# Autodesk Inventor assembly: Expansor
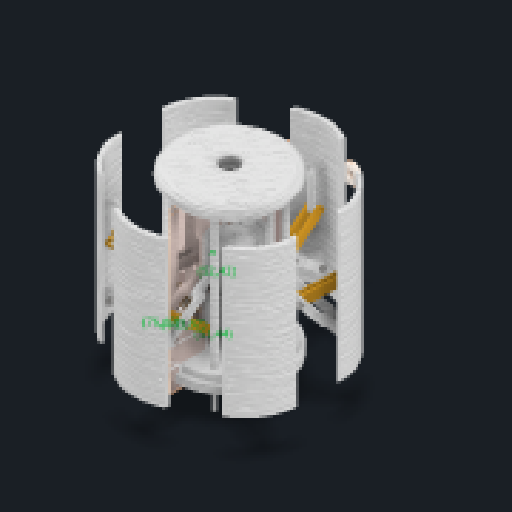
[picture p0: Inventor's stored thumbnail of the model, 512x512]
Saved by Autodesk Inventor 2025.3 (Build 293356030, 356C)
## iProperties
Created: 2024-12-25
Part Number: Expansor
Document SubType Name: Assembly
Designer: Usuario
Mass: 1399.4 g
Surface Area: 2444.05 cm^2
Volume: 493.018 cm^3
Density: 2.83844 g/cm^3
Author: Usuario
## Documents named in this file (19)
- C:\Users\santa\OneDrive - Universidad de los Andes\Robocol\Flotador\V3\Expansor.iam
- C:\Users\santa\OneDrive - Universidad de los Andes\Robocol\Flotador\V3\Expansor\Clavija.ipt
- C:\Users\santa\OneDrive - Universidad de los Andes\Robocol\Flotador\V3\Expansor\Columnas.ipt
- C:\Users\santa\OneDrive - Universidad de los Andes\Robocol\Flotador\V3\Expansor\Corredera I.ipt
- C:\Users\santa\OneDrive - Universidad de los Andes\Robocol\Flotador\V3\Expansor\Corredera II.ipt
- C:\Users\santa\OneDrive - Universidad de los Andes\Robocol\Flotador\V3\Expansor\Corredor.ipt
- C:\Users\santa\OneDrive - Universidad de los Andes\Robocol\Flotador\V3\Expansor\Paletas.ipt
- C:\Users\santa\OneDrive - Universidad de los Andes\Robocol\Flotador\V3\Expansor\Soporte.ipt
- C:\Users\santa\OneDrive - Universidad de los Andes\Robocol\Flotador\V3\Expansor\Tapa.ipt
- C:\Users\santa\OneDrive - Universidad de los Andes\Robocol\Flotador\Downloads\screw nut 8mm\screw nut 8mm.ipt
- C:\Users\santa\OneDrive\Documents\Inventor\Content Center Files\R2025\es-ES\ANSI B18.16.3M(2)\ANSI B18.16.3M - Property Class 5 and 10 - Metric M3 x 0.5 Tipo de metal.ipt
- C:\Users\santa\OneDrive\Documents\Inventor\Content Center Files\R2025\es-ES\AS 1420\AS 1420 - 1973 - M3 x 16.ipt
- C:\Users\santa\OneDrive - Universidad de los Andes\Robocol\Flotador\Downloads\688zz-bearing-2.snapshot.2\688ZZ Bearing\688ZZ Bearing Assembly\688ZZ Bearing Assembly\688ZZ Bearing Assembly.iam
- C:\Users\santa\OneDrive - Universidad de los Andes\Robocol\Flotador\V3\Expansor\AIP\FEA\exazi096o.fins
- C:\Users\santa\OneDrive - Universidad de los Andes\Robocol\Flotador\V3\Expansor\AIP\FEA\exazi096o.fsat
- C:\Users\santa\OneDrive - Universidad de los Andes\Robocol\Flotador\V3\Expansor\AIP\FEA\exazi096o.ftes
- C:\Users\santa\OneDrive - Universidad de los Andes\Robocol\Flotador\V3\Expansor\AIP\FEA\exazi096o.fwiz
- C:\Users\santa\OneDrive - Universidad de los Andes\Robocol\Flotador\V3\Expansor\AIP\FEA\exazi09pc.fmsh
- C:\Users\santa\OneDrive - Universidad de los Andes\Robocol\Flotador\V3\Expansor\AIP\FEA\exazi09pd.fres
## Components (83 placed, 12 different names)
1. Corredor:1 — ANIMAR, De rotación:5, Rígido:3, Simetría:1, Coincidencia:5, Simetría:2
2. Soporte:1 — Nivelación:1, Coincidencia:1, Nivelación:2, Rígido:1, ANIMAR, De rotación:3, Simetría:1, Simetría:2
3. Tapa:1 — Coincidencia:34, De rotación:6, Coincidencia:35
4. screw nut 8mm:1 — Rígido:3
5. 688ZZ Bearing Assembly:1 [sub-assembly] — De rotación:6
6. Tuerca hexagonal autofrenada - Acero Métrico Property Class 5 and 10 - Metric M3 x 0.5 Tipo de metal:2 — Coincidencia:10, Coincidencia:11
7. Tuerca hexagonal autofrenada - Acero Métrico Property Class 5 and 10 - Metric M3 x 0.5 Tipo de metal:4 — Coincidencia:28, Coincidencia:29
8. Tuerca hexagonal autofrenada - Acero Métrico Property Class 5 and 10 - Metric M3 x 0.5 Tipo de metal:3 — Coincidencia:14, Coincidencia:15
9. AS 1420 - Métrico M3 x 16:3 — Coincidencia:12, Coincidencia:13
10. AS 1420 - Métrico M3 x 16:4 — Coincidencia:26, Coincidencia:27
11. Tuerca hexagonal autofrenada - Acero Métrico Property Class 5 and 10 - Metric M3 x 0.5 Tipo de metal:5 — Coincidencia:32, Coincidencia:33
12. AS 1420 - Métrico M3 x 16:2 — Coincidencia:30, Coincidencia:31
13. Tuerca hexagonal autofrenada - Acero Métrico Property Class 5 and 10 - Metric M3 x 0.5 Tipo de metal:1 — Insertar:1
14. Columnas:1 — Rígido:1, Coincidencia:35
15. Corredera II:1 — De rotación:3, Coincidencia:3, Tangente:1, Coincidencia:7, Coincidencia:8, Coincidencia:9, Coincidencia:26, Coincidencia:27, Coincidencia:28, Coincidencia:29
16. Corredera I:1 — De rotación:5, Coincidencia:3, Coincidencia:6, Insertar:1, Coincidencia:11, Coincidencia:12, Coincidencia:13, Coincidencia:14, Coincidencia:15, Coincidencia:30, Coincidencia:31, Coincidencia:32, Coincidencia:33
17. Paletas:1 — Coincidencia:6, Tangente:1, Coincidencia:7
18. Clavija:1 — Coincidencia:8, Coincidencia:9, Coincidencia:10
19. Tuerca hexagonal autofrenada - Acero Métrico Property Class 5 and 10 - Metric M3 x 0.5 Tipo de metal:6
20. Tuerca hexagonal autofrenada - Acero Métrico Property Class 5 and 10 - Metric M3 x 0.5 Tipo de metal:7
21. Tuerca hexagonal autofrenada - Acero Métrico Property Class 5 and 10 - Metric M3 x 0.5 Tipo de metal:8
22. AS 1420 - Métrico M3 x 16:5
23. AS 1420 - Métrico M3 x 16:6
24. Tuerca hexagonal autofrenada - Acero Métrico Property Class 5 and 10 - Metric M3 x 0.5 Tipo de metal:9
25. AS 1420 - Métrico M3 x 16:7
26. Tuerca hexagonal autofrenada - Acero Métrico Property Class 5 and 10 - Metric M3 x 0.5 Tipo de metal:10
27. Columnas:2
28. Corredera II:2
29. Corredera I:2
30. Paletas:2
31. Clavija:2
32. Tuerca hexagonal autofrenada - Acero Métrico Property Class 5 and 10 - Metric M3 x 0.5 Tipo de metal:11
33. Tuerca hexagonal autofrenada - Acero Métrico Property Class 5 and 10 - Metric M3 x 0.5 Tipo de metal:12
34. Tuerca hexagonal autofrenada - Acero Métrico Property Class 5 and 10 - Metric M3 x 0.5 Tipo de metal:13
35. AS 1420 - Métrico M3 x 16:8
36. AS 1420 - Métrico M3 x 16:9
37. Tuerca hexagonal autofrenada - Acero Métrico Property Class 5 and 10 - Metric M3 x 0.5 Tipo de metal:14
38. AS 1420 - Métrico M3 x 16:10
39. Tuerca hexagonal autofrenada - Acero Métrico Property Class 5 and 10 - Metric M3 x 0.5 Tipo de metal:15
40. Columnas:3
41. Corredera II:3
42. Corredera I:3
43. Paletas:3
44. Clavija:3
45. Tuerca hexagonal autofrenada - Acero Métrico Property Class 5 and 10 - Metric M3 x 0.5 Tipo de metal:16
46. Tuerca hexagonal autofrenada - Acero Métrico Property Class 5 and 10 - Metric M3 x 0.5 Tipo de metal:17
47. Tuerca hexagonal autofrenada - Acero Métrico Property Class 5 and 10 - Metric M3 x 0.5 Tipo de metal:18
48. AS 1420 - Métrico M3 x 16:11
49. AS 1420 - Métrico M3 x 16:12
50. Tuerca hexagonal autofrenada - Acero Métrico Property Class 5 and 10 - Metric M3 x 0.5 Tipo de metal:19
51. AS 1420 - Métrico M3 x 16:13
52. Tuerca hexagonal autofrenada - Acero Métrico Property Class 5 and 10 - Metric M3 x 0.5 Tipo de metal:20
53. Columnas:4
54. Corredera II:4
55. Corredera I:4
56. Paletas:4
57. Clavija:4
58. Tuerca hexagonal autofrenada - Acero Métrico Property Class 5 and 10 - Metric M3 x 0.5 Tipo de metal:21
59. Tuerca hexagonal autofrenada - Acero Métrico Property Class 5 and 10 - Metric M3 x 0.5 Tipo de metal:22
60. Tuerca hexagonal autofrenada - Acero Métrico Property Class 5 and 10 - Metric M3 x 0.5 Tipo de metal:23
61. AS 1420 - Métrico M3 x 16:14
62. AS 1420 - Métrico M3 x 16:15
63. Tuerca hexagonal autofrenada - Acero Métrico Property Class 5 and 10 - Metric M3 x 0.5 Tipo de metal:24
64. AS 1420 - Métrico M3 x 16:16
65. Tuerca hexagonal autofrenada - Acero Métrico Property Class 5 and 10 - Metric M3 x 0.5 Tipo de metal:25
66. Columnas:5
67. Corredera II:5
68. Corredera I:5
69. Paletas:5
70. Clavija:5
71. Tuerca hexagonal autofrenada - Acero Métrico Property Class 5 and 10 - Metric M3 x 0.5 Tipo de metal:26
72. Tuerca hexagonal autofrenada - Acero Métrico Property Class 5 and 10 - Metric M3 x 0.5 Tipo de metal:27
73. Tuerca hexagonal autofrenada - Acero Métrico Property Class 5 and 10 - Metric M3 x 0.5 Tipo de metal:28
74. AS 1420 - Métrico M3 x 16:17
75. AS 1420 - Métrico M3 x 16:18
76. Tuerca hexagonal autofrenada - Acero Métrico Property Class 5 and 10 - Metric M3 x 0.5 Tipo de metal:29
77. AS 1420 - Métrico M3 x 16:19
78. Tuerca hexagonal autofrenada - Acero Métrico Property Class 5 and 10 - Metric M3 x 0.5 Tipo de metal:30
79. Columnas:6
80. Corredera II:6
81. Corredera I:6
82. Paletas:6
83. Clavija:6
## Component patterns: (6 elements, first: Tuerca hexagonal autofrenada - Acero Métrico Property Class 5 and 10 - Metric M3 x 0.5 Tipo de metal:2 + Tuerca hexagonal autofrenada - Acero Métrico Property Class 5 and 10 - Metric M3 x 0.5 Tipo de metal:4 + Tuerca hexagonal autofrenada - Acero Métrico Property Class 5 and 10 - Metric M3 x 0.5 Tipo de metal:3 + AS 1420 - Métrico M3 x 16:3 + AS 1420 - Métrico M3 x 16:4 + Tuerca hexagonal autofrenada - Acero Métrico Property Class 5 and 10 - Metric M3 x 0.5 Tipo de metal:5 + AS 1420 - Métrico M3 x 16:2 + Tuerca hexagonal autofrenada - Acero Métrico Property Class 5 and 10 - Metric M3 x 0.5 Tipo de metal:1 + Columnas:1 + Corredera II:1 + Corredera I:1 + Paletas:1 + Clavija:1)
## Relationships (35: Mate 23, RevoluteJoint 3, Flush 2, WeldJoint 2, Symmetry 2, CylindricalJoint 1, Tangent 1, Insert 1)
- Nivelación:1 [Flush]: Soporte:1
- Coincidencia:1 [Mate]: Soporte:1
- Nivelación:2 [Flush]: Soporte:1
- Rígido:1 [WeldJoint]: Soporte:1 ↔ Columnas:1
- ANIMAR [CylindricalJoint]: Corredor:1 ↔ Soporte:1
- De rotación:3 [RevoluteJoint]: Soporte:1 ↔ Corredera II:1
- De rotación:5 [RevoluteJoint]: Corredor:1 ↔ Corredera I:1
- Rígido:3 [WeldJoint]: Corredor:1 ↔ screw nut 8mm:1
- Simetría:1 [Symmetry]: Corredor:1 ↔ Soporte:1
- Coincidencia:3 [Mate]: Corredera II:1 ↔ Corredera I:1
- Coincidencia:5 [Mate]: Corredor:1
- Simetría:2 [Symmetry]: Corredor:1 ↔ Soporte:1
- Coincidencia:6 [Mate]: Corredera I:1 ↔ Paletas:1
- Tangente:1: Corredera II:1 ↔ Paletas:1
- Coincidencia:7 [Mate]: Corredera II:1 ↔ Paletas:1
- Coincidencia:8 [Mate]: Corredera II:1 ↔ Clavija:1
- Coincidencia:9 [Mate]: Corredera II:1 ↔ Clavija:1
- Insertar:1: Tuerca hexagonal autofrenada - Acero Métrico Property Class 5 and 10 - Metric M3 x 0.5 Tipo de metal:1 ↔ Corredera I:1
- Coincidencia:10 [Mate]: Tuerca hexagonal autofrenada - Acero Métrico Property Class 5 and 10 - Metric M3 x 0.5 Tipo de metal:2 ↔ Clavija:1
- Coincidencia:11 [Mate]: Tuerca hexagonal autofrenada - Acero Métrico Property Class 5 and 10 - Metric M3 x 0.5 Tipo de metal:2 ↔ Corredera I:1
- Coincidencia:12 [Mate]: AS 1420 - Métrico M3 x 16:3 ↔ Corredera I:1
- Coincidencia:13 [Mate]: AS 1420 - Métrico M3 x 16:3 ↔ Corredera I:1
- Coincidencia:14 [Mate]: Tuerca hexagonal autofrenada - Acero Métrico Property Class 5 and 10 - Metric M3 x 0.5 Tipo de metal:3 ↔ Corredera I:1
- Coincidencia:15 [Mate]: Tuerca hexagonal autofrenada - Acero Métrico Property Class 5 and 10 - Metric M3 x 0.5 Tipo de metal:3 ↔ Corredera I:1
- Coincidencia:26 [Mate]: AS 1420 - Métrico M3 x 16:4 ↔ Corredera II:1
- Coincidencia:27 [Mate]: AS 1420 - Métrico M3 x 16:4 ↔ Corredera II:1
- Coincidencia:28 [Mate]: Tuerca hexagonal autofrenada - Acero Métrico Property Class 5 and 10 - Metric M3 x 0.5 Tipo de metal:4 ↔ Corredera II:1
- Coincidencia:29 [Mate]: Tuerca hexagonal autofrenada - Acero Métrico Property Class 5 and 10 - Metric M3 x 0.5 Tipo de metal:4 ↔ Corredera II:1
- Coincidencia:30 [Mate]: AS 1420 - Métrico M3 x 16:2 ↔ Corredera I:1
- Coincidencia:31 [Mate]: AS 1420 - Métrico M3 x 16:2 ↔ Corredera I:1
- Coincidencia:32 [Mate]: Tuerca hexagonal autofrenada - Acero Métrico Property Class 5 and 10 - Metric M3 x 0.5 Tipo de metal:5 ↔ Corredera I:1
- Coincidencia:33 [Mate]: Tuerca hexagonal autofrenada - Acero Métrico Property Class 5 and 10 - Metric M3 x 0.5 Tipo de metal:5 ↔ Corredera I:1
- Coincidencia:34 [Mate]: Tapa:1
- De rotación:6 [RevoluteJoint]: Tapa:1 ↔ 688ZZ Bearing Assembly:1
- Coincidencia:35 [Mate]: Tapa:1 ↔ Columnas:1
